# Autodesk Inventor assembly: distance_short
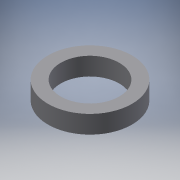
[picture p0: Inventor's stored thumbnail of the model, 180x180]
Saved by Autodesk Inventor 2019.3 (Build 233278000, 278)
## iProperties
Created: 2020-08-27
Part Number: distance_short
Material: Generisch
Document SubType Name: Assembly
Designer: Nicolas Frick
Author: Nicolas Frick
## Documents named in this file (2)
- C:\Users\Nicolas Frick\Sync\OneDrive\airhockeybot\mechanical_design\common_cad_parts\print_models\distance_short.iam
- C:\Users\Nicolas Frick\Sync\OneDrive\airhockeybot\mechanical_design\inventor\distance_short.ipt
## Components (1 placed, 1 different names)
1. distance_short:1 — Passend:1, Passend:2
## Relationships (2: Mate 2)
- Passend:1 [Mate]: distance_short:1
- Passend:2 [Mate]: distance_short:1
